# Autodesk Inventor assembly: крепление_мотора_для_шестерни
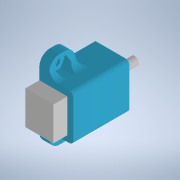
[picture p0: Inventor's stored thumbnail of the model, 180x180]
Saved by Autodesk Inventor 2021.1 (Build 251245010, 245A)
## iProperties
Created: 2023-02-11
Part Number: крепление_мотора_для_шестерни
Document SubType Name: Assembly
Designer: zmoze
Author: zmoze
## Documents named in this file (3)
- C:\Users\zmoze\OneDrive\Рабочий стол\GrabCAD\Smile_2022-2023\крепление_мотора_для_шестерни.iam
- C:\Users\zmoze\OneDrive\Рабочий стол\GrabCAD\Smile_2022-2023\крепление мотора для шестерни..ipt
- C:\Users\zmoze\OneDrive\Рабочий стол\GrabCAD\Smile_2022-2023\мотор_для_шестерни.ipt
## Components (2 placed, 2 different names)
1. крепление мотора для шестерни.:1 — Заподлицо:1, Совмещение:1, Совмещение:2
2. мотор_для_шестерни:1 — Заподлицо:1, Совмещение:1, Совмещение:2
## Relationships (3: Mate 2, Flush 1)
- Заподлицо:1 [Flush]: крепление мотора для шестерни.:1 ↔ мотор_для_шестерни:1
- Совмещение:1 [Mate]: крепление мотора для шестерни.:1 ↔ мотор_для_шестерни:1
- Совмещение:2 [Mate]: крепление мотора для шестерни.:1 ↔ мотор_для_шестерни:1
